# Autodesk Inventor assembly: Table_foot
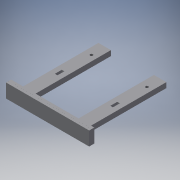
[picture p0: Inventor's stored thumbnail of the model, 180x180]
Saved by Autodesk Inventor 2019.4 (Build 234330000, 330)
## iProperties
Created: 2019-12-14
Part Number: Table_foot
Document SubType Name: Assembly
Designer: fabfarm
Author: fabfarm
## Documents named in this file (3)
- D:\Users\fabfarm\Documents\Saw table\Table_foot.iam
- D:\Users\fabfarm\Documents\Saw table\table_foot.ipt
- D:\Users\fabfarm\Documents\Saw table\table_bottont.ipt
## Components (6 placed, 2 different names)
1. table_bottont:1 — Mate:1, Mate:2, Flush:6, Flush:7, Mate:4, Mate:10
2. table_foot:1 — Flush:1, Mate:1, Mate:6, Flush:10, Flush:11
3. table_foot:2 — Flush:1, Mate:3, Flush:8, Flush:9, Mate:4, Mate:9
4. table_bottont:2 — Mate:2, Flush:6, Flush:7, Mate:8, Mate:9
5. table_foot:3 — Mate:3, Flush:8, Flush:9
6. table_foot:4 — Mate:6, Flush:10, Flush:11, Mate:8, Mate:10
## Relationships (15: Mate 8, Flush 7)
- Flush:1: table_foot:1 ↔ table_foot:2
- Mate:1: table_bottont:1 ↔ table_foot:1
- Mate:2: table_bottont:1 ↔ table_bottont:2
- Flush:6: table_bottont:1 ↔ table_bottont:2
- Flush:7: table_bottont:1 ↔ table_bottont:2
- Mate:3: table_foot:2 ↔ table_foot:3
- Flush:8: table_foot:2 ↔ table_foot:3
- Flush:9: table_foot:2 ↔ table_foot:3
- Mate:4: table_bottont:1 ↔ table_foot:2
- Mate:6: table_foot:1 ↔ table_foot:4
- Flush:10: table_foot:1 ↔ table_foot:4
- Flush:11: table_foot:1 ↔ table_foot:4
- Mate:8: table_bottont:2 ↔ table_foot:4
- Mate:9: table_foot:2 ↔ table_bottont:2
- Mate:10: table_bottont:1 ↔ table_foot:4
